# Autodesk Inventor assembly: Assembly1
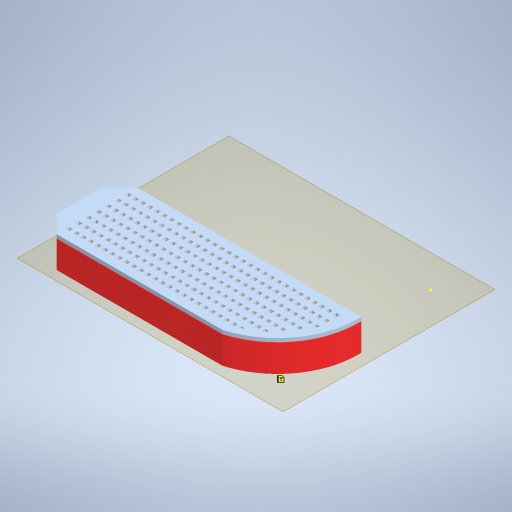
[picture p0: Inventor's stored thumbnail of the model, 512x512]
Saved by Autodesk Inventor 2024 (Build 280153000, 153)
## iProperties
Created: 2023-11-10
Part Number: Assembly1
Document SubType Name: Assembly
Designer: furqa
Author: furqa
## Documents named in this file (4)
- C:\Users\furqa\Desktop\P2\Individual Submissions\Assembly1.iam
- C:\Users\furqa\Desktop\P2\Individual Submissions\Box.ipt
- C:\Users\furqa\Desktop\P2\Individual Submissions\Cover_1.ipt
- C:\Users\furqa\Downloads\bonesaw\Tool-2 (Bone Saw).ipt
## Components (3 placed, 3 different names)
1. Box:1 — Mate:1, Mate:2, Mate:3
2. Cover_1:1 — Mate:1, Mate:2
3. Tool-2 (Bone Saw):1 — Mate:3
## Relationships (3: Mate 3)
- Mate:1: Box:1 ↔ Cover_1:1
- Mate:2: Box:1 ↔ Cover_1:1
- Mate:3 (5.08 mm): Box:1 ↔ Tool-2 (Bone Saw):1
## Named parameters: Finish10_Area = 33.7474, Finish1_Area = 124.712, Finish2_Area = 0.565487, Finish3_Area = 102.809, Finish4_Area = 33.7474, Finish5_Area = 5.00852, Finish6_Area = 27.4366, Finish7_Area = 20.3431, Finish8_Area = 11.1525, Finish9_Area = 33.7474
note: some values were not read from the file. Shown as the stored number, unit unknown: "Finish10_Area", "Finish1_Area", "Finish2_Area", "Finish3_Area", "Finish4_Area", "Finish5_Area", "Finish6_Area", "Finish7_Area", "Finish8_Area", "Finish9_Area".
